# Autodesk Inventor assembly: F_Foot
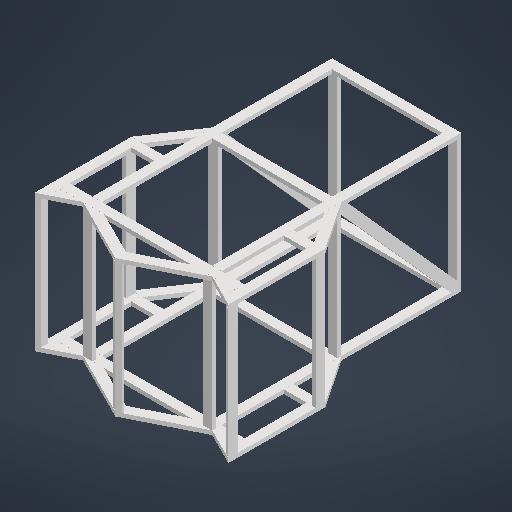
[picture p0: Inventor's stored thumbnail of the model, 512x512]
Saved by Autodesk Inventor 2026 (Build 300175000, 175)
## iProperties
Created: 2025-09-08
Part Number: F_Foot
Document SubType Name: Assembly
Designer: trott
Author: trott
## Documents named in this file (13)
- C:\Users\trott\Documents\UofSC-ASME-Tiger-Burn-Design-2025\CAD\Legs\Front Foot\F_Foot.iam
- C:\Users\trott\Documents\UofSC-ASME-Tiger-Burn-Design-2025\CAD\Legs\Front Foot\2x4x48.ipt
- C:\Users\trott\Documents\UofSC-ASME-Tiger-Burn-Design-2025\CAD\Legs\Front Foot\2x4x41.ipt
- C:\Users\trott\Documents\UofSC-ASME-Tiger-Burn-Design-2025\CAD\Legs\Front Foot\2x4x65.ipt
- C:\Users\trott\Documents\UofSC-ASME-Tiger-Burn-Design-2025\CAD\Legs\Front Foot\2x4x8.5.ipt
- C:\Users\trott\Documents\UofSC-ASME-Tiger-Burn-Design-2025\CAD\Legs\Front Foot\S_2x4x36.ipt
- C:\Users\trott\Documents\UofSC-ASME-Tiger-Burn-Design-2025\CAD\Legs\Front Foot\S_2x4x9.503.ipt
- C:\Users\trott\Documents\UofSC-ASME-Tiger-Burn-Design-2025\CAD\Legs\Front Foot\S_2x4x26.833.ipt
- C:\Users\trott\Documents\UofSC-ASME-Tiger-Burn-Design-2025\CAD\Legs\Front Foot\S2_2x4x48.ipt
- C:\Users\trott\Documents\UofSC-ASME-Tiger-Burn-Design-2025\CAD\Legs\Front Foot\S_2x4x48.ipt
- C:\Users\trott\Documents\UofSC-ASME-Tiger-Burn-Design-2025\CAD\Legs\Front Foot\S_2x4x21.633.ipt
- C:\Users\trott\Documents\UofSC-ASME-Tiger-Burn-Design-2025\CAD\Head\2x4x89.ipt
- C:\Users\trott\Documents\UofSC-ASME-Tiger-Burn-Design-2025\CAD\Legs\Front Foot\S_2x4x64.444.ipt
## Components (43 placed, 12 different names)
1. 2x4x48:7 — Mate:17, Flush:23, Flush:24
2. 2x4x48:8 — Mate:18, Flush:25, Flush:26
3. S2_2x4x48:1 — Mate:19, Flush:27, Flush:28
4. S_2x4x48:1
5. S_2x4x48:2
6. 2x4x48:9 — Mate:25, Flush:39, Mate:26
7. 2x4x48:10 — Mate:27, Mate:28, Flush:40, Mate:34
8. 2x4x41:3 — Mate:29, Flush:41, Flush:42
9. 2x4x41:4 — Mate:30, Flush:43, Flush:44
10. S_2x4x64.444:1 — Mate:31, Mate:32, Flush:45
11. S_2x4x64.444:2 — Mate:33, Mate:34, Mate:35
12. 2x4x48:2 — Flush:31, Flush:41, Flush:43, Mate:33
13. 2x4x48:3
14. 2x4x48:4 — Mate:20, Mate:32, Flush:45
15. 2x4x48:5 — Flush:32, Mate:22, Flush:33
16. S_2x4x21.633:1
17. S_2x4x21.633:2
18. S_2x4x21.633:3
19. S_2x4x21.633:4 — Mate:20, Flush:29
20. S_2x4x26.833:2 — Mate:14, Mate:15, Flush:20, Flush:27
21. S_2x4x26.833:1 — Mate:12, Mate:13, Flush:19, Mate:14, Mate:19, Flush:28
22. 2x4x65:1 — Mate:6, Flush:13, Mate:7, Flush:15, Mate:9, Mate:11, Mate:12, Flush:19, Mate:15, Flush:20, Mate:21, Flush:30, Flush:32, Mate:23, Flush:34
23. S_2x4x36:1 — Mate:6, Flush:13, Flush:14, Mate:8, Flush:17, Mate:17, Flush:23, Flush:24
24. S_2x4x9.503:1 — Mate:8, Flush:17, Mate:9, Mate:13
25. 2x4x89:1 — Mate:21, Flush:30, Flush:31, Flush:35, Flush:36, Mate:27, Mate:28, Flush:40, Mate:30, Flush:44, Mate:35
26. 2x4x8.5:1 — Flush:14
27. 2x4x89:2 — Mate:23, Flush:33, Flush:34, Mate:24, Flush:37, Flush:38, Mate:25, Flush:39, Mate:26
28. 2x4x8.5:2 — Flush:16
29. S_2x4x36:2 — Mate:7, Flush:15, Flush:16, Mate:10, Flush:18, Mate:18, Flush:25, Flush:26, Flush:29
30. S_2x4x9.503:2 — Mate:10, Mate:11, Flush:18, Mate:22
31. 2x4x41:1 — Mate:24, Flush:35, Flush:36, Flush:37, Flush:38
32. S_2x4x26.833:3
33. S_2x4x26.833:4
34. 2x4x65:2
35. S_2x4x36:3
36. S_2x4x9.503:3
37. 2x4x89:3 — Mate:29, Flush:42
38. 2x4x8.5:3
39. 2x4x89:4 — Mate:31
40. 2x4x8.5:4
41. S_2x4x36:4
42. S_2x4x9.503:4
43. 2x4x41:2
## Component patterns: (4 elements, first: 2x4x48:2), (2 elements, first: S_2x4x21.633:1 + S_2x4x21.633:2), (2 elements, first: S_2x4x26.833:2 + S_2x4x26.833:1 + 2x4x65:1 + S_2x4x36:1 + S_2x4x9.503:1 + 2x4x89:1 + 2x4x8.5:1 + 2x4x89:2 + 2x4x8.5:2 + S_2x4x36:2 + S_2x4x9.503:2 + 2x4x41:1)
## Relationships (60: Flush 31, Mate 29)
- Mate:6: 2x4x65:1 ↔ S_2x4x36:1
- Flush:13: 2x4x65:1 ↔ S_2x4x36:1
- Flush:14: S_2x4x36:1 ↔ 2x4x8.5:1
- Mate:7: 2x4x65:1 ↔ S_2x4x36:2
- Flush:15: 2x4x65:1 ↔ S_2x4x36:2
- Flush:16: 2x4x8.5:2 ↔ S_2x4x36:2
- Mate:8: S_2x4x36:1 ↔ S_2x4x9.503:1
- Flush:17: S_2x4x36:1 ↔ S_2x4x9.503:1
- Mate:9: 2x4x65:1 ↔ S_2x4x9.503:1
- Mate:10: S_2x4x36:2 ↔ S_2x4x9.503:2
- Mate:11: 2x4x65:1 ↔ S_2x4x9.503:2
- Flush:18: S_2x4x36:2 ↔ S_2x4x9.503:2
- Mate:12: S_2x4x26.833:1 ↔ 2x4x65:1
- Mate:13: S_2x4x26.833:1 ↔ S_2x4x9.503:1
- Flush:19: S_2x4x26.833:1 ↔ 2x4x65:1
- Mate:14: S_2x4x26.833:2 ↔ S_2x4x26.833:1
- Mate:15: S_2x4x26.833:2 ↔ 2x4x65:1
- Flush:20: S_2x4x26.833:2 ↔ 2x4x65:1
- Mate:17: 2x4x48:7 ↔ S_2x4x36:1
- Flush:23: 2x4x48:7 ↔ S_2x4x36:1
- Flush:24: 2x4x48:7 ↔ S_2x4x36:1
- Mate:18: 2x4x48:8 ↔ S_2x4x36:2
- Flush:25: 2x4x48:8 ↔ S_2x4x36:2
- Flush:26: 2x4x48:8 ↔ S_2x4x36:2
- Mate:19: S2_2x4x48:1 ↔ S_2x4x26.833:1
- Flush:27: S2_2x4x48:1 ↔ S_2x4x26.833:2
- Flush:28: S2_2x4x48:1 ↔ S_2x4x26.833:1
- Mate:20: 2x4x48:4 ↔ S_2x4x21.633:4
- Flush:29: S_2x4x21.633:4 ↔ S_2x4x36:2
- Mate:21: 2x4x65:1 ↔ 2x4x89:1
- Flush:30: 2x4x65:1 ↔ 2x4x89:1
- Flush:31: 2x4x48:2 ↔ 2x4x89:1
- Flush:32: 2x4x48:5 ↔ 2x4x65:1
- Mate:22: 2x4x48:5 ↔ S_2x4x9.503:2
- Mate:23: 2x4x65:1 ↔ 2x4x89:2
- Flush:33: 2x4x48:5 ↔ 2x4x89:2
- Flush:34: 2x4x65:1 ↔ 2x4x89:2
- Mate:24: 2x4x89:2 ↔ 2x4x41:1
- Flush:35: 2x4x89:1 ↔ 2x4x41:1
- Flush:36: 2x4x89:1 ↔ 2x4x41:1
- Flush:37: 2x4x89:2 ↔ 2x4x41:1
- Flush:38: 2x4x89:2 ↔ 2x4x41:1
- Mate:25: 2x4x48:9 ↔ 2x4x89:2
- Flush:39: 2x4x48:9 ↔ 2x4x89:2
- Mate:26: 2x4x48:9 ↔ 2x4x89:2
- Mate:27: 2x4x48:10 ↔ 2x4x89:1
- Mate:28: 2x4x48:10 ↔ 2x4x89:1
- Flush:40: 2x4x48:10 ↔ 2x4x89:1
- Mate:29: 2x4x41:3 ↔ 2x4x89:3
- Flush:41: 2x4x41:3 ↔ 2x4x48:2
- Flush:42: 2x4x41:3 ↔ 2x4x89:3
- Mate:30: 2x4x41:4 ↔ 2x4x89:1
- Flush:43: 2x4x41:4 ↔ 2x4x48:2
- Flush:44: 2x4x41:4 ↔ 2x4x89:1
- Mate:31: S_2x4x64.444:1 ↔ 2x4x89:4
- Mate:32: S_2x4x64.444:1 ↔ 2x4x48:4
- Flush:45: S_2x4x64.444:1 ↔ 2x4x48:4
- Mate:33: S_2x4x64.444:2 ↔ 2x4x48:2
- Mate:34: 2x4x48:10 ↔ S_2x4x64.444:2
- Mate:35: S_2x4x64.444:2 ↔ 2x4x89:1
